# Autodesk Inventor assembly: 742a 2.1 Intake Arm
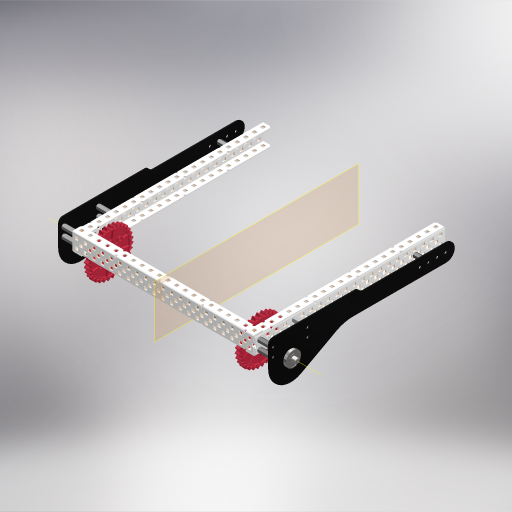
[picture p0: Inventor's stored thumbnail of the model, 512x512]
Saved by Autodesk Inventor 2024 (Build 280153000, 153)
## iProperties
Created: 2023-10-21
Part Number: 742a 2.1 Intake Arm
Document SubType Name: Assembly
Designer: aaron
Author: aaron
## Documents named in this file (10)
- C:\Users\aaron\Documents\Inventor\TritonRobotics\library\Subsystems\742a 2.1 Intake Arm.iam
- C:\Users\aaron\Documents\Inventor\TritonRobotics\library\VEX Library\Structure\C-Channels\Aluminum 1x2x1\1x2x1x21 Aluminum.ipt
- C:\Users\aaron\Documents\Inventor\TritonRobotics\library\Stock Material\Plates New\Intake Arm.ipt
- C:\Users\aaron\Documents\Inventor\TritonRobotics\library\VEX Library\Structure\C-Channels\Aluminum 1x2x1\1x2x1x22 Aluminum.ipt
- C:\Users\aaron\Documents\Inventor\TritonRobotics\library\VEX Library\Structure\Standoff\Standoff .75.ipt
- C:\Users\aaron\Documents\Inventor\TritonRobotics\library\VEX Library\Structure\Standoff.ipt
- C:\Users\aaron\Documents\Inventor\TritonRobotics\library\VEX Library\Motion\HS Shaft\bearing.ipt
- C:\Users\aaron\Documents\Inventor\TritonRobotics\library\VEX Library\Motion\HS Shaft\13in hs shaft.ipt
- C:\Users\aaron\Documents\Inventor\TritonRobotics\library\VEX Library\Motion\New Sprockets\32T.ipt
- C:\Users\aaron\Documents\Inventor\TritonRobotics\library\VEX Library\Motion\New Sprockets\8T.ipt
## Components (22 placed, 8 different names)
1. 1x2x1x21 Aluminum:3 — Mate:1, Mate:2, Mate:4
2. Intake Arm:1 — Mate:5, Mate:6, Mate:10, Mate:18, Mate:19, Mate:20, Mate:21, Mate:22, Mate:23, Mate:25, Mate:28, Mate:29, Symmetry:1
3. 1x2x1x22 Aluminum:1 — Mate:2, Mate:3, Mate:5, Mate:6, Mate:10, Mate:24
4. 1x2x1x22 Aluminum:2 — Mate:1, Mate:3, Mate:4, Mate:7, Mate:8, Mate:9
5. Intake Arm:2 — Mate:7, Mate:8, Mate:9, Mate:11, Mate:12, Mate:13, Mate:14, Mate:15, Mate:16, Mate:17, Mate:26, Mate:27, Mate:30, Mate:31, Symmetry:1
6. Standoff .75:1 — Mate:11, Mate:13
7. Standoff .75:2 — Mate:12, Mate:14
8. Standoff .75:3 — Flush:1, Mate:15, Mate:16
9. Standoff .75:4 — Flush:1, Mate:17
10. Standoff .75:5 — Flush:2, Mate:18, Mate:19
11. Standoff .75:6 — Flush:2, Mate:20
12. Standoff .75:7 — Mate:23
13. Standoff .75:8 — Mate:21, Mate:22
14. Standoff .75:9 — Mate:24, Mate:25
15. Standoff .75:10 — Mate:26, Mate:27
16. bearing:1 — Mate:30, Mate:31, Mate:37
17. bearing:2 — Mate:28, Mate:29, Mate:32, Flush:4, Mate:38
18. 13in hs shaft:1 — Mate:32, Flush:4, Mate:33, Mate:34, Mate:35, Mate:36
19. 32T:1 — Mate:33, Mate:39
20. 32T:2 — Mate:34, Mate:39
21. 8T:1 — Mate:36, Mate:37
22. 8T:2 — Mate:35, Mate:38
## Relationships (44: Mate 39, Flush 4, Symmetry 1)
- Mate:1: 1x2x1x21 Aluminum:3 ↔ 1x2x1x22 Aluminum:2
- Mate:2: 1x2x1x21 Aluminum:3 ↔ 1x2x1x22 Aluminum:1
- Mate:3: 1x2x1x22 Aluminum:1 ↔ 1x2x1x22 Aluminum:2
- Mate:4: 1x2x1x21 Aluminum:3 ↔ 1x2x1x22 Aluminum:2
- Mate:5: Intake Arm:1 ↔ 1x2x1x22 Aluminum:1
- Mate:6: Intake Arm:1 ↔ 1x2x1x22 Aluminum:1
- Mate:7: 1x2x1x22 Aluminum:2 ↔ Intake Arm:2
- Mate:8: 1x2x1x22 Aluminum:2 ↔ Intake Arm:2
- Mate:9 (19.05 mm): 1x2x1x22 Aluminum:2 ↔ Intake Arm:2
- Mate:10 (19.05 mm): Intake Arm:1 ↔ 1x2x1x22 Aluminum:1
- Mate:11: Intake Arm:2 ↔ Standoff .75:1
- Mate:12: Intake Arm:2 ↔ Standoff .75:2
- Mate:13: Intake Arm:2 ↔ Standoff .75:1
- Mate:14: Intake Arm:2 ↔ Standoff .75:2
- Flush:1: Standoff .75:3 ↔ Standoff .75:4
- Mate:15: Intake Arm:2 ↔ Standoff .75:3
- Mate:16: Intake Arm:2 ↔ Standoff .75:3
- Mate:17: Intake Arm:2 ↔ Standoff .75:4
- Flush:2: Standoff .75:5 ↔ Standoff .75:6
- Mate:18: Intake Arm:1 ↔ Standoff .75:5
- Mate:19: Intake Arm:1 ↔ Standoff .75:5
- Mate:20: Intake Arm:1 ↔ Standoff .75:6
- [Flush]: Standoff .75:7 ↔ Standoff .75:8
- Mate:21: Intake Arm:1 ↔ Standoff .75:8
- Mate:22: Intake Arm:1 ↔ Standoff .75:8
- Mate:23: Intake Arm:1 ↔ Standoff .75:7
- Mate:24: 1x2x1x22 Aluminum:1 ↔ Standoff .75:9
- Mate:25: Intake Arm:1 ↔ Standoff .75:9
- Mate:26: Intake Arm:2 ↔ Standoff .75:10
- Mate:27: Intake Arm:2 ↔ Standoff .75:10
- Mate:28: Intake Arm:1 ↔ bearing:2
- Mate:29: Intake Arm:1 ↔ bearing:2
- Mate:30: Intake Arm:2 ↔ bearing:1
- Mate:31: Intake Arm:2 ↔ bearing:1
- Mate:32: bearing:2 ↔ 13in hs shaft:1
- Flush:4 (-6.35 mm): bearing:2 ↔ 13in hs shaft:1
- Mate:33: 13in hs shaft:1 ↔ 32T:1
- Mate:34: 13in hs shaft:1 ↔ 32T:2
- Mate:35: 13in hs shaft:1 ↔ 8T:2
- Mate:36: 13in hs shaft:1 ↔ 8T:1
- Mate:37: bearing:1 ↔ 8T:1
- Mate:38: bearing:2 ↔ 8T:2
- Mate:39 (209.55 mm): 32T:1 ↔ 32T:2
- Symmetry:1: Intake Arm:1 ↔ Intake Arm:2
## Named parameters: d28_d24 = 0 mm
